# Autodesk Inventor assembly: Assembly
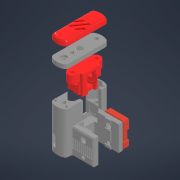
[picture p0: Inventor's stored thumbnail of the model, 180x180]
Saved by Autodesk Inventor 2022.1 (Build 261234000, 234)
## iProperties
Created: 2021-10-02
Part Number: Assembly
Document SubType Name: Assembly
Designer: Rama
Author: Rama
## Documents named in this file (7)
- C:\Users\Rama\Desktop\GitHub\Voron-2-Mods\Front_Idlers\CAD\Assembly.iam
- C:\Users\Rama\Desktop\GitHub\Voron-2-Mods\Front_Idlers\CAD\Front-Idlers_Housing.ipt
- C:\Users\Rama\Desktop\GitHub\Voron-2-Mods\Front_Idlers\CAD\Front-Idlers_Housing-Cover.ipt
- C:\Users\Rama\Desktop\GitHub\Voron-2-Mods\Front_Idlers\CAD\Front-Idlers_Inlet.ipt
- C:\Users\Rama\Desktop\GitHub\Voron-2-Mods\Front_Idlers\CAD\Front-Idlers_Z-Belt-Clamp-Upper.ipt
- C:\Users\Rama\Desktop\GitHub\Voron-2-Mods\Misumi_RBPB5\CAD\Src\6x3 Magnet.ipt
- C:\Users\Rama\Desktop\GitHub\Voron-2-Mods\Front_Idlers\CAD\Covers\Cover_Round.ipt
## Components (7 placed, 6 different names)
1. Front-Idlers_Housing:1 — Passend:1, Passend:2, Passend:3, Passend:9, Passend:10, Passend:11
2. Front-Idlers_Housing-Cover:1 — Passend:3, Passend:4, Passend:5, Fluchtend:1, Passend:7, Passend:8
3. Front-Idlers_Inlet:1 — Passend:1, Passend:2, Passend:4
4. Front-Idlers_Z-Belt-Clamp-Upper:1 — Passend:9, Passend:10, Passend:11
5. 6x3 Magnet:1 — Passend:5, Fluchtend:1
6. 6x3 Magnet:2 — Passend:6, Fluchtend:2
7. Cover_Round:1 — Passend:6, Fluchtend:2, Passend:7, Passend:8
## Relationships (13: Mate 11, Flush 2)
- Passend:1 [Mate]: Front-Idlers_Housing:1 ↔ Front-Idlers_Inlet:1
- Passend:2 [Mate]: Front-Idlers_Housing:1 ↔ Front-Idlers_Inlet:1
- Passend:3 [Mate]: Front-Idlers_Housing:1 ↔ Front-Idlers_Housing-Cover:1
- Passend:4 [Mate]: Front-Idlers_Housing-Cover:1 ↔ Front-Idlers_Inlet:1
- Passend:5 [Mate]: Front-Idlers_Housing-Cover:1 ↔ 6x3 Magnet:1
- Fluchtend:1 [Flush]: Front-Idlers_Housing-Cover:1 ↔ 6x3 Magnet:1
- Passend:6 [Mate]: 6x3 Magnet:2 ↔ Cover_Round:1
- Fluchtend:2 [Flush]: 6x3 Magnet:2 ↔ Cover_Round:1
- Passend:7 [Mate]: Front-Idlers_Housing-Cover:1 ↔ Cover_Round:1
- Passend:8 [Mate]: Front-Idlers_Housing-Cover:1 ↔ Cover_Round:1
- Passend:9 [Mate]: Front-Idlers_Housing:1 ↔ Front-Idlers_Z-Belt-Clamp-Upper:1
- Passend:10 [Mate]: Front-Idlers_Housing:1 ↔ Front-Idlers_Z-Belt-Clamp-Upper:1
- Passend:11 [Mate]: Front-Idlers_Housing:1 ↔ Front-Idlers_Z-Belt-Clamp-Upper:1
